(part 1 of 3)
# Autodesk Inventor assembly: Assembly1
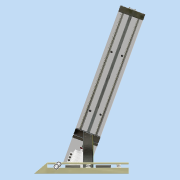
[picture p0: Inventor's stored thumbnail of the model, 180x180]
Saved by Autodesk Inventor 2021 (Build 250183000, 183)
## iProperties
Created: 2024-03-13
Part Number: Assembly1
Document SubType Name: Assembly
Designer: Nokia
Author: Nokia
## Documents named in this file (48)
- C:\Users\Nokia\Desktop\KP22\KP2\Assembly1.iam
- C:\Users\Nokia\Desktop\KP22\KP2\Plattform-Oberteil.ipt
- C:\Users\Nokia\Desktop\KP22\KP2\Spindel.ipt
- C:\Users\Nokia\Documents\Inventor\Content Center Files\R2021\en-US\DIN 711 SKF\DIN 711 SKF - SKF 51108.ipt
- C:\Users\Nokia\Documents\Inventor\Content Center Files\R2021\en-US\DIN 981\DIN 981 - KM 6.ipt
- C:\Users\Nokia\Documents\Inventor\Content Center Files\R2021\en-US\DIN 5406 Type MB_MBL (- DIN 981)\DIN 5406 - MB6.ipt
- C:\Users\Nokia\Documents\Inventor\Content Center Files\R2021\en-US\DIN 625 SKF(5)\DIN 625 SKF - SKF 6206-2RS1.ipt
- C:\Users\Nokia\Desktop\KP22\KP2\Festlagertopf.ipt
- C:\Users\Nokia\Desktop\KP22\KP2\Deckel.ipt
- C:\Users\Nokia\Desktop\KP22\KP2\Deckelscheibe.ipt
- C:\Users\Nokia\Desktop\KP22\KP2\Plattform-Unterteil.ipt
- C:\Users\Nokia\Desktop\KP22\KP2\Verbindungsplatte.ipt
- C:\Users\Nokia\Documents\Inventor\Content Center Files\R2021\en-US\DIN 625 SKF(5)\DIN 625 SKF - SKF 6005-2RSH.ipt
- C:\Users\Nokia\Documents\Inventor\Content Center Files\R2021\en-US\DIN 5406 Type MB_MBL (- DIN 981)\DIN 5406 - MB5.ipt
- C:\Users\Nokia\Documents\Inventor\Content Center Files\R2021\en-US\DIN 981\DIN 981 - KM 5.ipt
- C:\Users\Nokia\Desktop\KP22\KP2\Loslagertopf.ipt
- C:\Users\Nokia\Desktop\KP22\KP2\Verfahrschlitten.ipt
- C:\Users\Nokia\Desktop\KP22\KP2\Federwellen-Gleitlager.ipt
- C:\Users\Nokia\Desktop\KP22\KP2\Federführungswellen.ipt
- C:\Users\Nokia\Desktop\KP22\KP2\Hülle des Plattform-Oberteils.ipt
- C:\Users\Nokia\Desktop\KP22\KP2\Hülle des Plattform-Unterteils.ipt
- C:\Users\Nokia\Documents\Inventor\Content Center Files\R2021\en-US\DIN 931-1\DIN 931-1 - M6 x 30.ipt
- C:\Users\Nokia\Documents\Inventor\Content Center Files\R2021\en-US\DIN 125-1  B\DIN 125-1 - B 6,4.ipt
- C:\Users\Nokia\Documents\Inventor\Content Center Files\R2021\en-US\DIN 931-1\DIN 931-1 - M8 x 50.ipt
- C:\Users\Nokia\Documents\Inventor\Content Center Files\R2021\en-US\DIN 125-1  B\DIN 125-1 - B 8,4.ipt
- C:\Users\Nokia\Documents\Inventor\Content Center Files\R2021\en-US\DIN 931-1\DIN 931-1 - M6 x 50.ipt
- C:\Users\Nokia\Desktop\KP22\KP2\Gewindemutter.ipt
- C:\Users\Nokia\Documents\Inventor\Content Center Files\R2021\en-US\DIN 125-1  B\DIN 125-1 - B 5,3.ipt
- C:\Users\Nokia\Documents\Inventor\Content Center Files\R2021\en-US\DIN 931-1\DIN 931-1 - M5 x 25.ipt
- C:\Users\Nokia\Desktop\KP22\KP2\Führung.ipt
- C:\Users\Nokia\Documents\Inventor\Content Center Files\R2021\en-US\DIN 931-1\DIN 931-1 - M5 x 50.ipt
- C:\Users\Nokia\Desktop\KP22\KP2\Führungsgleitlager.ipt
- C:\Users\Nokia\Desktop\KP22\KP2\Schutzpuffer.ipt
- C:\Users\Nokia\Desktop\KP22\KP2\Grundplatte.ipt
- C:\Users\Nokia\Documents\Inventor\Content Center Files\R2021\en-US\DIN 125-1  B\DIN 125-1 - B 13.ipt
- C:\Users\Nokia\Documents\Inventor\Content Center Files\R2021\en-US\DIN 931-1\DIN 931-1 - M12 x 70.ipt
- C:\Users\Nokia\Desktop\KP22\KP2\Elektromotor.ipt
- C:\Users\Nokia\Desktop\KP22\KP2\Ausgleichskupplung.iam
- C:\Users\Nokia\Documents\Inventor\Content Center Files\R2021\en-US\DIN 912\DIN 912 - M12 x 1,75 x 50 x 45,625.ipt
- C:\Users\Nokia\Documents\Inventor\Content Center Files\R2021\en-US\DIN 6915\DIN 6915 - M12.ipt
- C:\Users\Nokia\Documents\Inventor\Content Center Files\R2021\en-US\DIN 6885-1 A\DIN 6885 - A 4 x 4 x 12.ipt
- C:\Users\Nokia\Documents\Inventor\Content Center Files\R2021\en-US\DIN EN ISO 4026\DIN EN ISO 4026 - M8 x 10.ipt
- C:\Users\Nokia\Desktop\KP22\KP2\Rubber Kupplung.ipt
- C:\Users\Nokia\Desktop\KP22\KP2\Elektrischer Schalter.ipt
- C:\Users\Nokia\Desktop\KP22\KP2\Wand.ipt
- C:\Users\Nokia\Desktop\KP22\KP2\Compress Spring11.ipt
- C:\Users\Nokia\Documents\Inventor\Content Center Files\R2021\en-US\DIN 931-1\DIN 931-1 - M12 x 55.ipt
- C:\Users\Nokia\Documents\Inventor\Content Center Files\R2021\en-US\DIN 931-1\DIN 931-1 - M8 x 45.ipt
## Components (277 placed, 47 different names)
1. Plattform-Oberteil:1 — Mate:60, Mate:61, Mate:62, Mate:63, Mate:64, Mate:65, Mate:66, Mate:67, Mate:68, Mate:69, Mate:70, Mate:71, Mate:85, Mate:86, Mate:87, Mate:88, Mate:89, Mate:90, Mate:91, Mate:92, Mate:93, Mate:94, Mate:95, Mate:96, Mate:97, Angle:13, Angle:14, Angle:15, Angle:16, Angle:17, Mate:122, Mate:123, Mate:124, Mate:125, Mate:126, Mate:127, Mate:146, Mate:147, Mate:153, Mate:154, Mate:191, Mate:192, Mate:193, Mate:194, Mate:195, Mate:196, Mate:197, Mate:198, Mate:199, Mate:200, Mate:201, Mate:202, Mate:203, Mate:204, Mate:205, Mate:206, Mate:207, Mate:223, Mate:224, Mate:225, Mate:226, Mate:227, Mate:497, Mate:645, Mate:646, Mate:647, Mate:648, Mate:649, Mate:650
2. DIN 711 SKF SKF 51108:1 — Mate:10, Mate:11, Mate:18, Mate:655
3. DIN 625 SKF- with two RS1 seals SKF 6206-2RS1:1 — Mate:3, Mate:4, Mate:20, Mate:651, Mate:654
4. Spindel:1 — Mate:3, Mate:4, Mate:10, Mate:11, Mate:13, Mate:14, Mate:17, Mate:19, Mate:21, Mate:46, Mate:47, Mate:48, Mate:50, Angle:5, Mate:52, Mate:55, Mate:548, Mate:551, Mate:552, Mate:553, Angle:21, Mate:654, Mate:655, Mate:656
5. DIN 981 KM 6:1 — Mate:16, Mate:17, Angle:2
6. DIN 5406 Type MB/MBL (->DIN 981) MB6:1 — Mate:13, Mate:14, Mate:16, Mate:651
7. Festlagertopf:1 — Mate:18, Mate:19, Angle:2, Angle:4, Mate:272, Mate:321, Mate:322, Mate:323, Mate:324, Mate:337, Mate:338, Mate:339, Mate:340, Mate:341, Mate:342, Mate:343, Mate:344, Mate:345, Mate:346, Mate:347, Mate:348, Flush:4, Mate:447, Mate:473, Mate:474, Mate:475, Mate:476, Mate:477, Mate:478, Mate:479, Angle:21
8. Deckel:1 — Mate:20, Mate:21, Mate:28, Mate:29, Mate:30, Mate:31, Mate:32, Mate:33, Mate:266, Mate:267, Mate:268, Mate:269, Mate:270, Mate:271
9. Deckelscheibe:1 — Mate:22, Mate:23, Mate:31
10. Deckelscheibe:2 — Mate:22, Mate:23, Mate:28
11. Deckelscheibe:3 — Mate:33
12. Deckelscheibe:4 — Mate:30
13. Deckelscheibe:5 — Mate:32
14. Deckelscheibe:6 — Mate:29
15. Plattform-Unterteil:1 — Mate:36, Mate:37, Mate:38, Mate:72, Mate:73, Mate:74, Mate:75, Mate:76, Mate:77, Mate:78, Mate:79, Mate:80, Mate:81, Mate:82, Mate:83, Mate:116, Mate:117, Mate:118, Mate:119, Mate:120, Mate:121, Mate:134, Mate:135, Mate:136, Mate:137, Mate:138, Mate:139, Mate:236, Mate:237, Mate:238, Mate:239, Mate:242, Mate:243, Mate:497, Mate:617, Mate:618, Flush:10, Flush:11, Flush:12, Flush:13, Angle:136, Angle:154, Angle:156, Angle:158, Angle:162, Angle:164, Angle:176
16. Verbindungsplatte:1 — Mate:36, Mate:37, Mate:38, Mate:53, Mate:56, Mate:57, Mate:58, Mate:59, Mate:240, Mate:241, Mate:252, Mate:253, Mate:254, Mate:255, Mate:256, Mate:257, Mate:258, Mate:259
17. DIN 625 SKF- with two RS1 seals SKF 6005-2RSH:1 — Mate:40, Mate:41, Mate:46, Mate:47, Mate:652, Mate:656
18. DIN 981 KM 5:1 — Mate:51, Angle:5, Mate:52
19. DIN 5406 Type MB/MBL (->DIN 981) MB5:1 — Mate:48, Mate:50, Mate:51, Mate:652
20. Loslagertopf:1 — Mate:40, Mate:41, Angle:4, Angle:6, Mate:492, Mate:493, Mate:494, Mate:495, Mate:657
21. Verfahrschlitten:1 — Mate:53, Angle:6, Mate:55, Mate:56, Mate:57, Mate:58, Mate:59, Mate:275, Mate:276, Mate:277, Mate:278, Mate:279, Mate:301, Mate:302, Mate:303, Mate:304, Mate:305, Mate:311, Mate:313, Mate:314, Mate:315, Mate:316, Mate:389, Mate:390, Mate:393, Mate:394, Mate:404, Mate:405, Mate:406, Mate:407, Mate:408, Mate:409, Mate:410, Mate:411, Mate:412, Mate:413, Mate:414, Mate:415, Mate:418, Mate:420, Mate:421, Mate:422, Mate:423, Mate:424, Mate:425, Mate:426, Mate:427, Mate:428, Mate:429, Mate:430, Mate:501, Mate:502, Angle:18, Angle:19, Flush:5, Flush:6, Flush:7, Flush:8, Mate:504, Angle:84, Angle:85, Angle:102, Angle:103, Angle:107, Angle:112, Angle:117, Angle:122, Angle:126, Angle:127
22. Federwellen-Gleitlager:1 — Mate:60, Mate:66
23. Federwellen-Gleitlager:2 — Mate:61, Mate:67
24. Federwellen-Gleitlager:3 — Mate:65, Mate:71
25. Federwellen-Gleitlager:4 — Mate:64, Mate:70
26. Federwellen-Gleitlager:5 — Mate:62, Mate:69
27. Federwellen-Gleitlager:6 — Mate:63, Mate:68
28. Federwellen-Gleitlager:7 — Mate:72, Mate:79, Mate:85
29. Federwellen-Gleitlager:8 — Mate:75, Mate:81
30. Federwellen-Gleitlager:9 — Mate:74, Mate:80
31. Federwellen-Gleitlager:10 — Mate:77, Mate:82, Mate:496
32. Federwellen-Gleitlager:11 — Mate:76, Mate:83
33. Federwellen-Gleitlager:12 — Mate:73, Mate:78
34. Federführungswellen:1 — Mate:87, Mate:95, Mate:115, Mate:129, Mate:143, Mate:208, Mate:209, Mate:210, Mate:644
35. Federführungswellen:2 — Mate:86, Mate:96, Mate:114, Mate:128, Mate:142, Mate:149, Mate:639
36. Federführungswellen:3 — Mate:88, Mate:97, Mate:112, Mate:131, Mate:144, Mate:211, Mate:212, Mate:213, Mate:643
37. Federführungswellen:4 — Mate:89, Mate:94, Mate:113, Mate:130, Mate:141, Mate:214, Mate:215, Mate:216, Mate:640
38. Federführungswellen:5 — Mate:90, Mate:92, Mate:98, Mate:99, Mate:132, Mate:140, Mate:217, Mate:218, Mate:219, Mate:496, Mate:641
39. Federführungswellen:6 — Mate:91, Mate:93, Mate:111, Mate:133, Mate:145, Mate:220, Mate:221, Mate:222, Mate:642
40. DIN 981 KM 6:3 — Mate:101, Mate:102, Angle:8, Mate:116, Angle:155
41. DIN 981 KM 6:4 — Mate:98, Mate:100, Angle:7, Mate:117, Angle:157
42. DIN 981 KM 6:6 — Mate:99, Mate:100, Angle:7, Angle:156, Angle:157
43. DIN 981 KM 6:7 — Mate:101, Mate:102, Angle:8, Mate:111, Angle:17, Angle:154, Angle:155
44. DIN 981 KM 6:8 — Mate:121, Angle:163
45. DIN 981 KM 6:9 — Mate:114, Angle:13, Angle:162, Angle:163
46. DIN 981 KM 6:10 — Mate:119, Angle:159
47. DIN 981 KM 6:11 — Mate:112, Angle:16, Angle:158, Angle:159, Angle:160
48. DIN 981 KM 6:12 — Mate:118, Angle:161
49. DIN 981 KM 6:13 — Mate:113, Angle:15, Angle:160, Angle:161
50. DIN 981 KM 6:14 — Mate:120, Angle:165
51. DIN 981 KM 6:15 — Mate:115, Angle:14, Angle:164, Angle:165
52. Hülle des Plattform-Oberteils:1 — Mate:125, Mate:130
53. Hülle des Plattform-Oberteils:2 — Mate:126, Mate:132
54. Hülle des Plattform-Oberteils:3 — Mate:127, Mate:133
55. Hülle des Plattform-Oberteils:4 — Mate:124, Mate:131
56. Hülle des Plattform-Oberteils:5 — Mate:122, Mate:128
57. Hülle des Plattform-Oberteils:6 — Mate:123, Mate:129
58. Hülle des Plattform-Unterteils:1 — Mate:134, Mate:142
59. Hülle des Plattform-Unterteils:2 — Mate:135, Mate:143
60. Hülle des Plattform-Unterteils:3 — Mate:136, Mate:141
61. Hülle des Plattform-Unterteils:4 — Mate:137, Mate:144
62. Hülle des Plattform-Unterteils:5 — Mate:138, Mate:140
63. Hülle des Plattform-Unterteils:6 — Mate:139, Mate:145
64. DIN 125-1 B B 6,4:1 — Mate:146, Mate:147, Mate:148, Mate:150
65. DIN 931-1 - replaced by DIN EN 24014 M6 x 30:1 — Mate:148, Mate:149, Mate:150, Angle:141
66. DIN 125-1 B B 6,4:2 — Mate:153
67. DIN 931-1 - replaced by DIN EN 24014 M6 x 30:2 — Mate:154, Angle:139, Angle:140, Angle:141, Angle:142
68. DIN 125-1 B B 6,4:4 — Mate:197
69. DIN 931-1 - replaced by DIN EN 24014 M6 x 30:4 — Mate:212, Mate:225, Angle:147
70. DIN 125-1 B B 6,4:5 — Mate:202
71. DIN 931-1 - replaced by DIN EN 24014 M6 x 30:5 — Mate:217, Mate:227, Angle:148, Angle:150, Angle:151
72. DIN 125-1 B B 6,4:7 — Mate:198
73. DIN 931-1 - replaced by DIN EN 24014 M6 x 30:7 — Mate:215, Angle:142, Angle:143
74. DIN 125-1 B B 6,4:8 — Mate:200, Mate:224
75. DIN 931-1 - replaced by DIN EN 24014 M6 x 30:8 — Mate:214, Angle:143, Angle:144
76. DIN 125-1 B B 6,4:9 — Mate:204
77. DIN 931-1 - replaced by DIN EN 24014 M6 x 30:9 — Mate:220, Angle:153
78. DIN 125-1 B B 6,4:10 — Mate:195
79. DIN 931-1 - replaced by DIN EN 24014 M6 x 30:10 — Mate:213, Angle:145, Angle:146, Angle:148
80. DIN 125-1 B B 6,4:11 — Mate:196
81. DIN 931-1 - replaced by DIN EN 24014 M6 x 30:11 — Mate:211, Angle:146, Angle:147
82. DIN 125-1 B B 6,4:12 — Mate:206
83. DIN 931-1 - replaced by DIN EN 24014 M6 x 30:12 — Mate:222, Angle:151, Angle:152, Angle:153
84. DIN 125-1 B B 6,4:13 — Mate:201
85. DIN 931-1 - replaced by DIN EN 24014 M6 x 30:13 — Mate:218, Angle:184
86. DIN 125-1 B B 6,4:14 — Mate:205
87. DIN 931-1 - replaced by DIN EN 24014 M6 x 30:14 — Mate:221, Mate:226, Angle:152
88. DIN 125-1 B B 6,4:15 — Mate:203
89. DIN 931-1 - replaced by DIN EN 24014 M6 x 30:15 — Mate:219, Angle:150, Angle:184
90. DIN 125-1 B B 6,4:16 — Mate:192
91. DIN 931-1 - replaced by DIN EN 24014 M6 x 30:16 — Mate:210, Angle:138, Angle:139
92. DIN 125-1 B B 6,4:17 — Mate:194, Mate:207
93. DIN 931-1 - replaced by DIN EN 24014 M6 x 30:17 — Angle:140
94. DIN 125-1 B B 6,4:18 — Mate:199
95. DIN 931-1 - replaced by DIN EN 24014 M6 x 30:18 — Mate:216, Angle:144, Angle:145
96. DIN 125-1 B B 6,4:19 — Mate:191
97. DIN 931-1 - replaced by DIN EN 24014 M6 x 30:19 — Mate:208, Mate:223, Angle:136, Angle:137
98. DIN 125-1 B B 6,4:20 — Mate:193
99. DIN 931-1 - replaced by DIN EN 24014 M6 x 30:20 — Mate:209, Angle:137, Angle:138
100. DIN 931-1 - replaced by DIN EN 24014 M8 x 45:1 — Mate:228, Mate:229, Mate:243, Angle:175, Angle:180, Angle:181, Angle:182, Angle:183
101. DIN 125-1 B B 8,4:1 — Mate:228, Mate:229, Mate:236
102. DIN 931-1 - replaced by DIN EN 24014 M8 x 45:2 — Mate:242, Angle:175, Angle:181
103. DIN 125-1 B B 8,4:2 — Mate:238
104. DIN 931-1 - replaced by DIN EN 24014 M8 x 45:3 — Mate:240, Angle:183
105. DIN 125-1 B B 8,4:3 — Mate:239
106. DIN 931-1 - replaced by DIN EN 24014 M8 x 45:4 — Mate:241, Angle:182
107. DIN 125-1 B B 8,4:4 — Mate:237
108. DIN 931-1 - replaced by DIN EN 24014 M8 x 50:5 — Mate:259, Angle:178
109. DIN 125-1 B B 8,4:5 — Mate:255
110. DIN 931-1 - replaced by DIN EN 24014 M8 x 50:6 — Mate:258, Angle:179, Angle:180
111. DIN 125-1 B B 8,4:6 — Mate:254
112. DIN 931-1 - replaced by DIN EN 24014 M8 x 50:7 — Mate:257, Angle:177, Angle:178, Angle:179
113. DIN 125-1 B B 8,4:7 — Mate:253
114. DIN 931-1 - replaced by DIN EN 24014 M8 x 50:8 — Mate:256, Angle:176, Angle:177
115. DIN 125-1 B B 8,4:8 — Mate:252
116. DIN 931-1 - replaced by DIN EN 24014 M6 x 50:3 — Mate:270, Angle:32
117. DIN 125-1 B B 6,4:23 — Mate:268
118. DIN 931-1 - replaced by DIN EN 24014 M6 x 50:2 — Mate:269, Mate:272, Angle:33
119. DIN 125-1 B B 6,4:21 — Mate:266
120. DIN 931-1 - replaced by DIN EN 24014 M6 x 50:1 — Mate:271, Angle:28, Angle:31
121. DIN 125-1 B B 6,4:22 — Mate:267
122. DIN 931-1 - replaced by DIN EN 24014 M5 x 25:1 — Mate:279, Mate:312, Angle:111
123. DIN 125-1 B B 5,3:2 — Mate:280
124. Gewindemutter:1 — Mate:275, Mate:276, Mate:280, Mate:312, Mate:317, Mate:318, Mate:319, Mate:320
125. Gewindemutter:2 — Mate:277, Mate:278, Mate:306, Mate:307, Mate:308, Mate:309, Mate:310
126. DIN 931-1 - replaced by DIN EN 24014 M5 x 25:2 — Mate:320, Angle:109, Angle:111
127. DIN 125-1 B B 5,3:3 — Mate:316
128. DIN 931-1 - replaced by DIN EN 24014 M5 x 25:3 — Mate:318, Angle:108
129. DIN 125-1 B B 5,3:4 — Mate:315
130. DIN 931-1 - replaced by DIN EN 24014 M5 x 25:4 — Mate:308, Angle:126
131. DIN 125-1 B B 5,3:5 — Mate:305
132. DIN 931-1 - replaced by DIN EN 24014 M5 x 25:5 — Mate:319, Angle:107, Angle:108, Angle:109, Angle:110
133. DIN 125-1 B B 5,3:6 — Mate:313
134. DIN 931-1 - replaced by DIN EN 24014 M5 x 25:6 — Mate:307, Angle:125
135. DIN 125-1 B B 5,3:7 — Mate:304
136. DIN 931-1 - replaced by DIN EN 24014 M5 x 25:7 — Mate:317, Angle:110
137. DIN 125-1 B B 5,3:8 — Mate:314
138. DIN 931-1 - replaced by DIN EN 24014 M5 x 25:8 — Mate:309, Mate:311, Angle:124
139. DIN 125-1 B B 5,3:9 — Mate:301
140. DIN 931-1 - replaced by DIN EN 24014 M5 x 25:9 — Mate:310, Angle:123
141. DIN 125-1 B B 5,3:10 — Mate:302
142. DIN 931-1 - replaced by DIN EN 24014 M5 x 25:11 — Mate:306, Angle:122, Angle:123, Angle:124, Angle:125
143. DIN 125-1 B B 5,3:12 — Mate:303
144. Führung:1 — Mate:321, Mate:323, Mate:417, Mate:505, Mate:653
145. Führung:2 — Mate:322, Mate:324, Mate:391, Mate:416
146. DIN 931-1 - replaced by DIN EN 24014 M5 x 50:4 — Mate:345, Angle:25
147. DIN 125-1 B B 5,3:14 — Mate:337
148. DIN 931-1 - replaced by DIN EN 24014 M5 x 50:1 — Mate:347, Angle:30, Mate:653
149. DIN 125-1 B B 5,3:16 — Mate:338
150. DIN 931-1 - replaced by DIN EN 24014 M5 x 50:2 — Mate:348, Angle:29
151. DIN 125-1 B B 5,3:17 — Mate:340
152. DIN 931-1 - replaced by DIN EN 24014 M5 x 50:5 — Mate:343, Angle:26
153. DIN 125-1 B B 5,3:18 — Mate:342
154. DIN 931-1 - replaced by DIN EN 24014 M5 x 50:6 — Mate:344, Angle:27
155. DIN 125-1 B B 5,3:19 — Mate:339
156. DIN 931-1 - replaced by DIN EN 24014 M5 x 50:3 — Mate:346
157. DIN 125-1 B B 5,3:20 — Mate:341
158. DIN 931-1 - replaced by DIN EN 24014 M5 x 25:12 — Mate:438, Angle:104, Angle:105
159. DIN 125-1 B B 5,3:21 — Mate:421
160. Führungsgleitlager:1 — Mate:417, Mate:418, Mate:431, Mate:432, Mate:433, Mate:434, Mate:440
161. Führungsgleitlager:2 — Mate:415, Mate:416, Mate:420, Mate:435, Mate:436, Mate:437, Mate:438, Mate:439
162. Führungsgleitlager:3 — Mate:389, Mate:393, Mate:395, Mate:396, Mate:397, Mate:398, Mate:399, Mate:400, Mate:401, Mate:402, Mate:403, Mate:505
163. Führungsgleitlager:4 — Mate:390, Mate:391, Mate:394
164. DIN 931-1 - replaced by DIN EN 24014 M5 x 25:13 — Mate:437, Angle:103, Angle:106
165. DIN 125-1 B B 5,3:22 — Mate:428
166. DIN 931-1 - replaced by DIN EN 24014 M5 x 25:14 — Mate:410, Angle:128
167. DIN 125-1 B B 5,3:23 — Mate:401
168. DIN 931-1 - replaced by DIN EN 24014 M5 x 25:15 — Mate:413, Angle:118
169. DIN 125-1 B B 5,3:24 — Mate:396
170. DIN 931-1 - replaced by DIN EN 24014 M5 x 25:16 — Mate:409, Angle:130
171. DIN 125-1 B B 5,3:25 — Mate:404
172. DIN 931-1 - replaced by DIN EN 24014 M5 x 25:17 — Mate:435, Angle:105
173. DIN 125-1 B B 5,3:26 — Mate:424
174. DIN 931-1 - replaced by DIN EN 24014 M5 x 25:18 — Mate:408, Angle:121
175. DIN 125-1 B B 5,3:27 — Mate:400
176. DIN 931-1 - replaced by DIN EN 24014 M5 x 25:19 — Mate:405, Angle:119
177. DIN 125-1 B B 5,3:28 — Mate:398
178. DIN 931-1 - replaced by DIN EN 24014 M5 x 25:20 — Mate:407, Angle:117, Angle:118, Angle:119, Angle:120, Angle:121
179. DIN 125-1 B B 5,3:29 — Mate:399
180. DIN 931-1 - replaced by DIN EN 24014 M5 x 25:21 — Mate:412, Angle:129
181. DIN 125-1 B B 5,3:30 — Mate:403
182. DIN 931-1 - replaced by DIN EN 24014 M5 x 25:22 — Mate:406, Angle:120
183. DIN 125-1 B B 5,3:31 — Mate:402
184. DIN 931-1 - replaced by DIN EN 24014 M5 x 25:23 — Mate:411, Angle:131
185. DIN 125-1 B B 5,3:32 — Mate:397
186. DIN 931-1 - replaced by DIN EN 24014 M5 x 25:24 — Mate:439, Angle:102, Angle:104
187. DIN 125-1 B B 5,3:33 — Mate:427
188. DIN 931-1 - replaced by DIN EN 24014 M5 x 25:25 — Mate:436, Angle:106
189. DIN 125-1 B B 5,3:34 — Mate:422
190. DIN 931-1 - replaced by DIN EN 24014 M5 x 25:26 — Mate:432, Mate:504, Angle:115
191. DIN 125-1 B B 5,3:35 — Mate:430
192. DIN 931-1 - replaced by DIN EN 24014 M5 x 25:27 — Mate:433, Angle:116
193. DIN 125-1 B B 5,3:36 — Mate:423
194. DIN 931-1 - replaced by DIN EN 24014 M5 x 25:28 — Mate:414, Angle:127, Angle:128, Angle:129, Angle:130, Angle:131
195. DIN 125-1 B B 5,3:37 — Mate:395
196. DIN 931-1 - replaced by DIN EN 24014 M5 x 25:29 — Mate:434, Angle:113
197. DIN 125-1 B B 5,3:38 — Mate:425
198. DIN 931-1 - replaced by DIN EN 24014 M5 x 25:30 — Mate:440, Angle:112, Angle:113, Angle:114, Angle:115, Angle:116
199. DIN 125-1 B B 5,3:39 — Mate:429
200. DIN 931-1 - replaced by DIN EN 24014 M5 x 25:31 — Mate:431, Angle:114
201. DIN 125-1 B B 5,3:40 — Mate:426
202. Grundplatte:1 — Flush:4, Mate:447, Mate:465, Mate:466, Mate:467, Mate:468, Mate:469, Mate:470, Mate:471, Mate:472, Mate:488, Mate:489, Mate:490, Mate:491, Mate:499, Mate:500, Angle:20, Flush:9, Mate:520, Mate:521, Mate:522, Mate:523, Mate:524, Mate:525, Mate:531, Mate:532, Mate:546, Mate:547, Mate:619, Mate:628, Mate:629, Mate:630, Mate:631, Mate:632, Mate:633, Mate:634, Mate:635, Angle:25, Angle:26, Angle:27, Angle:28, Angle:29, Angle:30, Angle:31, Angle:32, Angle:33, Angle:34, Angle:35, Angle:36, Angle:37, Angle:38, Angle:39, Angle:40, Angle:41, Angle:42, Angle:43, Angle:44, Angle:45, Angle:86, Angle:87, Angle:88, Angle:89, Angle:90, Angle:91, Angle:92, Angle:93, Angle:94, Angle:95, Angle:96, Angle:97, Angle:166, Angle:167
203. DIN 931-1 - replaced by DIN EN 24014 M12 x 70:1 — Mate:478, Angle:92
204. DIN 125-1 B B 13:1 — Mate:465
205. DIN 931-1 - replaced by DIN EN 24014 M12 x 70:2 — Mate:500, Angle:91
206. DIN 125-1 B B 13:2 — Mate:466
207. DIN 931-1 - replaced by DIN EN 24014 M12 x 70:3 — Mate:473, Angle:97
208. DIN 125-1 B B 13:3 — Mate:467
209. DIN 931-1 - replaced by DIN EN 24014 M12 x 70:4 — Mate:474, Angle:96
210. DIN 125-1 B B 13:4 — Mate:468
211. DIN 931-1 - replaced by DIN EN 24014 M12 x 70:5 — Mate:475, Angle:95
212. DIN 125-1 B B 13:5 — Mate:469
213. DIN 931-1 - replaced by DIN EN 24014 M12 x 70:6 — Mate:476, Angle:94
214. DIN 125-1 B B 13:6 — Mate:470
215. DIN 931-1 - replaced by DIN EN 24014 M12 x 70:7 — Mate:477, Angle:93
216. DIN 125-1 B B 13:7 — Mate:471
217. DIN 931-1 - replaced by DIN EN 24014 M12 x 70:8 — Mate:479, Angle:90
218. DIN 125-1 B B 13:8 — Mate:472
219. DIN 931-1 - replaced by DIN EN 24014 M12 x 70:9 — Mate:494, Angle:88
220. DIN 125-1 B B 13:9 — Mate:489
221. DIN 931-1 - replaced by DIN EN 24014 M12 x 70:10 — Mate:492, Angle:86
222. DIN 125-1 B B 13:10 — Mate:488
223. DIN 931-1 - replaced by DIN EN 24014 M12 x 70:11 — Mate:493, Mate:499, Angle:82, Angle:83, Angle:87
224. DIN 125-1 B B 13:11 — Mate:490
225. DIN 931-1 - replaced by DIN EN 24014 M12 x 70:12 — Mate:495, Angle:89
226. DIN 125-1 B B 13:12 — Mate:491
227. Schutzpuffer:1 — Mate:502, Angle:18, Flush:5, Flush:6, Mate:657
228. Schutzpuffer:2 — Mate:501, Angle:19, Flush:7, Flush:8
229. Elektromotor:1 — Angle:20, Flush:9, Mate:526, Mate:527, Mate:528, Mate:529, Mate:530, Mate:533, Mate:534, Mate:535, Mate:536, Mate:537, Mate:538, Mate:539, Mate:547, Mate:548, Mate:549, Mate:550, Mate:636, Mate:637, Mate:638
230. Ausgleichskupplung:1 [sub-assembly] — Mate:549, Mate:550, Angle:22, Mate:561, Mate:562
231. DIN 912 - replaced by DIN EN ISO 4762 M12 x 50:1 — Mate:508, Mate:509, Mate:530, Mate:544, Angle:37
232. DIN 125-1 B B 13:13 — Mate:508, Mate:509, Mate:525
233. DIN 912 - replaced by DIN EN ISO 4762 M12 x 50:2 — Mate:529, Mate:543, Angle:39
234. DIN 125-1 B B 13:14 — Mate:524
235. DIN 912 - replaced by DIN EN ISO 4762 M12 x 50:3 — Mate:527, Mate:540, Angle:45
236. DIN 125-1 B B 13:15 — Mate:520, Mate:522
237. DIN 912 - replaced by DIN EN ISO 4762 M12 x 50:4 — Mate:533, Mate:545, Angle:38
238. DIN 125-1 B B 13:16 — Mate:532
239. DIN 912 - replaced by DIN EN ISO 4762 M12 x 50:5 — Mate:528, Mate:541, Angle:44
240. DIN 125-1 B B 13:17 — Mate:521, Mate:523
241. DIN 912 - replaced by DIN EN ISO 4762 M12 x 50:6 — Mate:526, Mate:542, Mate:546, Angle:43
242. DIN 125-1 B B 13:18 — Mate:531
243. DIN 125-1 B B 13:19 — Mate:539, Mate:541, Insert:5
244. DIN 125-1 B B 13:20 — Mate:538, Mate:542, Insert:4
245. DIN 125-1 B B 13:21 — Mate:537, Mate:543, Insert:1
246. DIN 125-1 B B 13:22 — Mate:536, Mate:540, Insert:6
247. DIN 125-1 B B 13:23 — Mate:535, Mate:545, Insert:3
248. DIN 125-1 B B 13:24 — Mate:534, Mate:544, Insert:2
249. DIN 6915 M12:1 — Insert:1, Angle:36
250. DIN 6915 M12:2 — Insert:2, Angle:35
251. DIN 6915 M12:3 — Insert:3, Angle:34
252. DIN 6915 M12:4 — Insert:4, Angle:42
253. DIN 6915 M12:5 — Insert:5, Angle:41
254. DIN 6915 M12:6 — Insert:6, Angle:40
255. DIN 6885-1 A A 4 x 4 x 12:2 — Mate:563, Mate:636, Mate:637, Mate:638, Angle:23
256. DIN 6885-1 A A 4 x 4 x 12:1 — Mate:551, Mate:552, Mate:553, Angle:22, Mate:564, Angle:24
257. DIN EN ISO 4026 M8 x 10:1 — Mate:557, Mate:559, Mate:562, Angle:83
258. DIN EN ISO 4026 M8 x 10:2 — Mate:558, Mate:560, Mate:561, Angle:82
259. Rubber Kupplung:1 — Mate:557, Mate:559, Mate:563, Angle:23
260. Rubber Kupplung:2 — Mate:558, Mate:560, Mate:564, Angle:24
261. Elektrischer Schalter:1 — Mate:617, Flush:11, Flush:13
262. Elektrischer Schalter:2 — Mate:618, Flush:10, Flush:12
263. Wand:1 — Mate:619
264. DIN 931-1 - replaced by DIN EN 24014 M12 x 55:4 — Mate:632, Angle:166
265. DIN 125-1 B B 13:26 — Mate:631
266. DIN 931-1 - replaced by DIN EN 24014 M12 x 55:3 — Mate:633, Angle:167
267. DIN 125-1 B B 13:25 — Mate:630
268. DIN 931-1 - replaced by DIN EN 24014 M12 x 55:1 — Mate:635, Angle:85
269. DIN 125-1 B B 13:28 — Mate:628
270. DIN 931-1 - replaced by DIN EN 24014 M12 x 55:2 — Mate:634, Angle:84
271. DIN 125-1 B B 13:27 — Mate:629
272. Compress Spring1:1 — Mate:639, Mate:645
273. Compress Spring1:2 — Mate:640, Mate:647
274. Compress Spring1:3 — Mate:641, Mate:648
275. Compress Spring1:4 — Mate:642, Mate:649
276. Compress Spring1:5 — Mate:643, Mate:650
277. Compress Spring1:6 — Mate:644, Mate:646
## Relationships (710: Mate 564, Angle 130, Flush 10, Insert 6)
- Mate:3: DIN 625 SKF- with two RS1 seals SKF 6206-2RS1:1 ↔ Spindel:1
- Mate:4: DIN 625 SKF- with two RS1 seals SKF 6206-2RS1:1 ↔ Spindel:1
- Mate:10: DIN 711 SKF SKF 51108:1 ↔ Spindel:1
- Mate:11: DIN 711 SKF SKF 51108:1 ↔ Spindel:1
- Mate:13: Spindel:1 ↔ DIN 5406 Type MB/MBL (->DIN 981) MB6:1
- Mate:14: Spindel:1 ↔ DIN 5406 Type MB/MBL (->DIN 981) MB6:1
- Mate:16: DIN 981 KM 6:1 ↔ DIN 5406 Type MB/MBL (->DIN 981) MB6:1
- Mate:17: Spindel:1 ↔ DIN 981 KM 6:1
- Mate:18: DIN 711 SKF SKF 51108:1 ↔ Festlagertopf:1
- Mate:19: Spindel:1 ↔ Festlagertopf:1
- Angle:2 (0 deg): DIN 981 KM 6:1 ↔ Festlagertopf:1
- Mate:20: DIN 625 SKF- with two RS1 seals SKF 6206-2RS1:1 ↔ Deckel:1
- Mate:21: Spindel:1 ↔ Deckel:1
- Mate:22: Deckelscheibe:1 ↔ Deckelscheibe:2
- Mate:23: Deckelscheibe:1 ↔ Deckelscheibe:2
- [Mate]: Deckelscheibe:3 ↔ Deckelscheibe:4
- [Mate]: Deckelscheibe:3 ↔ Deckelscheibe:4
- [Mate]: Deckelscheibe:5 ↔ Deckelscheibe:6
- [Mate]: Deckelscheibe:5 ↔ Deckelscheibe:6
- Mate:28: Deckel:1 ↔ Deckelscheibe:2
- Mate:29: Deckel:1 ↔ Deckelscheibe:6
- Mate:30: Deckel:1 ↔ Deckelscheibe:4
- Mate:31: Deckel:1 ↔ Deckelscheibe:1
- Mate:32: Deckel:1 ↔ Deckelscheibe:5
- Mate:33: Deckel:1 ↔ Deckelscheibe:3
- Mate:36: Plattform-Unterteil:1 ↔ Verbindungsplatte:1
- Mate:37: Plattform-Unterteil:1 ↔ Verbindungsplatte:1
- Mate:38: Plattform-Unterteil:1 ↔ Verbindungsplatte:1
- Mate:40: DIN 625 SKF- with two RS1 seals SKF 6005-2RSH:1 ↔ Loslagertopf:1
- Mate:41: DIN 625 SKF- with two RS1 seals SKF 6005-2RSH:1 ↔ Loslagertopf:1
- Angle:4 (0 deg): Festlagertopf:1 ↔ Loslagertopf:1
- Mate:46: Spindel:1 ↔ DIN 625 SKF- with two RS1 seals SKF 6005-2RSH:1
- Mate:47: Spindel:1 ↔ DIN 625 SKF- with two RS1 seals SKF 6005-2RSH:1
- Mate:48: Spindel:1 ↔ DIN 5406 Type MB/MBL (->DIN 981) MB5:1
- Mate:50: Spindel:1 ↔ DIN 5406 Type MB/MBL (->DIN 981) MB5:1
- Mate:51: DIN 981 KM 5:1 ↔ DIN 5406 Type MB/MBL (->DIN 981) MB5:1
- Angle:5 (0 deg): Spindel:1 ↔ DIN 981 KM 5:1
- Mate:52: Spindel:1 ↔ DIN 981 KM 5:1
- Mate:53: Verbindungsplatte:1 ↔ Verfahrschlitten:1
- Angle:6 (0 deg): Loslagertopf:1 ↔ Verfahrschlitten:1
- Mate:55: Spindel:1 ↔ Verfahrschlitten:1
- Mate:56: Verbindungsplatte:1 ↔ Verfahrschlitten:1
- Mate:57: Verbindungsplatte:1 ↔ Verfahrschlitten:1
- Mate:58: Verbindungsplatte:1 ↔ Verfahrschlitten:1
- Mate:59: Verbindungsplatte:1 ↔ Verfahrschlitten:1
- Mate:60: Plattform-Oberteil:1 ↔ Federwellen-Gleitlager:1
- Mate:61: Plattform-Oberteil:1 ↔ Federwellen-Gleitlager:2
- Mate:62: Plattform-Oberteil:1 ↔ Federwellen-Gleitlager:5
- Mate:63: Plattform-Oberteil:1 ↔ Federwellen-Gleitlager:6
- Mate:64: Plattform-Oberteil:1 ↔ Federwellen-Gleitlager:4
- Mate:65: Plattform-Oberteil:1 ↔ Federwellen-Gleitlager:3
- Mate:66: Plattform-Oberteil:1 ↔ Federwellen-Gleitlager:1
- Mate:67: Plattform-Oberteil:1 ↔ Federwellen-Gleitlager:2
- Mate:68: Plattform-Oberteil:1 ↔ Federwellen-Gleitlager:6
- Mate:69: Plattform-Oberteil:1 ↔ Federwellen-Gleitlager:5
- Mate:70: Plattform-Oberteil:1 ↔ Federwellen-Gleitlager:4
- Mate:71: Plattform-Oberteil:1 ↔ Federwellen-Gleitlager:3
- Mate:72: Plattform-Unterteil:1 ↔ Federwellen-Gleitlager:7
- Mate:73: Plattform-Unterteil:1 ↔ Federwellen-Gleitlager:12
- Mate:74: Plattform-Unterteil:1 ↔ Federwellen-Gleitlager:9
- Mate:75: Plattform-Unterteil:1 ↔ Federwellen-Gleitlager:8
- Mate:76: Plattform-Unterteil:1 ↔ Federwellen-Gleitlager:11
- Mate:77: Plattform-Unterteil:1 ↔ Federwellen-Gleitlager:10
- Mate:78: Plattform-Unterteil:1 ↔ Federwellen-Gleitlager:12
- Mate:79: Plattform-Unterteil:1 ↔ Federwellen-Gleitlager:7
- Mate:80: Plattform-Unterteil:1 ↔ Federwellen-Gleitlager:9
- Mate:81: Plattform-Unterteil:1 ↔ Federwellen-Gleitlager:8
- Mate:82: Plattform-Unterteil:1 ↔ Federwellen-Gleitlager:10
- Mate:83: Plattform-Unterteil:1 ↔ Federwellen-Gleitlager:11
- Mate:85: Plattform-Oberteil:1 ↔ Federwellen-Gleitlager:7
- Mate:86: Plattform-Oberteil:1 ↔ Federführungswellen:2
- Mate:87: Plattform-Oberteil:1 ↔ Federführungswellen:1
- Mate:88: Plattform-Oberteil:1 ↔ Federführungswellen:3
- Mate:89: Plattform-Oberteil:1 ↔ Federführungswellen:4
- Mate:90: Plattform-Oberteil:1 ↔ Federführungswellen:5
- Mate:91: Plattform-Oberteil:1 ↔ Federführungswellen:6
- Mate:92: Plattform-Oberteil:1 ↔ Federführungswellen:5
- Mate:93: Plattform-Oberteil:1 ↔ Federführungswellen:6
- Mate:94: Plattform-Oberteil:1 ↔ Federführungswellen:4
- Mate:95: Plattform-Oberteil:1 ↔ Federführungswellen:1
- Mate:96: Plattform-Oberteil:1 ↔ Federführungswellen:2
- Mate:97: Plattform-Oberteil:1 ↔ Federführungswellen:3
- Mate:98: Federführungswellen:5 ↔ DIN 981 KM 6:4
- Mate:99: Federführungswellen:5 ↔ DIN 981 KM 6:6
- Mate:100: DIN 981 KM 6:4 ↔ DIN 981 KM 6:6
- Angle:7 (0 deg): DIN 981 KM 6:4 ↔ DIN 981 KM 6:6
- Mate:101: DIN 981 KM 6:3 ↔ DIN 981 KM 6:7
- Mate:102: DIN 981 KM 6:3 ↔ DIN 981 KM 6:7
- Angle:8 (0 deg): DIN 981 KM 6:3 ↔ DIN 981 KM 6:7
- [Mate]: DIN 981 KM 6:8 ↔ DIN 981 KM 6:9
- [Mate]: DIN 981 KM 6:8 ↔ DIN 981 KM 6:9
- [Angle] (0 deg): DIN 981 KM 6:8 ↔ DIN 981 KM 6:9
- [Mate]: DIN 981 KM 6:10 ↔ DIN 981 KM 6:11
- [Mate]: DIN 981 KM 6:10 ↔ DIN 981 KM 6:11
- [Angle] (0 deg): DIN 981 KM 6:10 ↔ DIN 981 KM 6:11
- [Mate]: DIN 981 KM 6:12 ↔ DIN 981 KM 6:13
- [Mate]: DIN 981 KM 6:12 ↔ DIN 981 KM 6:13
- [Angle] (0 deg): DIN 981 KM 6:12 ↔ DIN 981 KM 6:13
- [Mate]: DIN 981 KM 6:14 ↔ DIN 981 KM 6:15
- [Mate]: DIN 981 KM 6:14 ↔ DIN 981 KM 6:15
- [Angle] (0 deg): DIN 981 KM 6:14 ↔ DIN 981 KM 6:15
- Mate:111: Federführungswellen:6 ↔ DIN 981 KM 6:7
- Mate:112: Federführungswellen:3 ↔ DIN 981 KM 6:11
- Mate:113: Federführungswellen:4 ↔ DIN 981 KM 6:13
- Mate:114: Federführungswellen:2 ↔ DIN 981 KM 6:9
- Mate:115: Federführungswellen:1 ↔ DIN 981 KM 6:15
- Angle:13 (0 deg): Plattform-Oberteil:1 ↔ DIN 981 KM 6:9
- Angle:14 (0 deg): Plattform-Oberteil:1 ↔ DIN 981 KM 6:15
- Angle:15 (0 deg): Plattform-Oberteil:1 ↔ DIN 981 KM 6:13
- Angle:16 (0 deg): Plattform-Oberteil:1 ↔ DIN 981 KM 6:11
- Angle:17 (0 deg): Plattform-Oberteil:1 ↔ DIN 981 KM 6:7
- Mate:116: Plattform-Unterteil:1 ↔ DIN 981 KM 6:3
- Mate:117: Plattform-Unterteil:1 ↔ DIN 981 KM 6:4
- Mate:118: Plattform-Unterteil:1 ↔ DIN 981 KM 6:12
- Mate:119: Plattform-Unterteil:1 ↔ DIN 981 KM 6:10
- Mate:120: Plattform-Unterteil:1 ↔ DIN 981 KM 6:14
- Mate:121: Plattform-Unterteil:1 ↔ DIN 981 KM 6:8
- Mate:122: Plattform-Oberteil:1 ↔ Hülle des Plattform-Oberteils:5
- Mate:123: Plattform-Oberteil:1 ↔ Hülle des Plattform-Oberteils:6
- Mate:124: Plattform-Oberteil:1 ↔ Hülle des Plattform-Oberteils:4
- Mate:125: Plattform-Oberteil:1 ↔ Hülle des Plattform-Oberteils:1
- Mate:126: Plattform-Oberteil:1 ↔ Hülle des Plattform-Oberteils:2
- Mate:127: Plattform-Oberteil:1 ↔ Hülle des Plattform-Oberteils:3
- Mate:128: Federführungswellen:2 ↔ Hülle des Plattform-Oberteils:5
- Mate:129: Federführungswellen:1 ↔ Hülle des Plattform-Oberteils:6
- Mate:130: Federführungswellen:4 ↔ Hülle des Plattform-Oberteils:1
- Mate:131: Federführungswellen:3 ↔ Hülle des Plattform-Oberteils:4
- Mate:132: Federführungswellen:5 ↔ Hülle des Plattform-Oberteils:2
- Mate:133: Federführungswellen:6 ↔ Hülle des Plattform-Oberteils:3
- Mate:134: Plattform-Unterteil:1 ↔ Hülle des Plattform-Unterteils:1
- Mate:135: Plattform-Unterteil:1 ↔ Hülle des Plattform-Unterteils:2
- Mate:136: Plattform-Unterteil:1 ↔ Hülle des Plattform-Unterteils:3
- Mate:137: Plattform-Unterteil:1 ↔ Hülle des Plattform-Unterteils:4
- Mate:138: Plattform-Unterteil:1 ↔ Hülle des Plattform-Unterteils:5
- Mate:139: Plattform-Unterteil:1 ↔ Hülle des Plattform-Unterteils:6
- Mate:140: Federführungswellen:5 ↔ Hülle des Plattform-Unterteils:5
- Mate:141: Federführungswellen:4 ↔ Hülle des Plattform-Unterteils:3
- Mate:142: Federführungswellen:2 ↔ Hülle des Plattform-Unterteils:1
- Mate:143: Federführungswellen:1 ↔ Hülle des Plattform-Unterteils:2
- Mate:144: Federführungswellen:3 ↔ Hülle des Plattform-Unterteils:4
- Mate:145: Federführungswellen:6 ↔ Hülle des Plattform-Unterteils:6
- Mate:146: Plattform-Oberteil:1 ↔ DIN 125-1 B B 6,4:1
- Mate:147: Plattform-Oberteil:1 ↔ DIN 125-1 B B 6,4:1
- Mate:148: DIN 125-1 B B 6,4:1 ↔ DIN 931-1 - replaced by DIN EN 24014 M6 x 30:1
- Mate:149: Federführungswellen:2 ↔ DIN 931-1 - replaced by DIN EN 24014 M6 x 30:1
- Mate:150: DIN 125-1 B B 6,4:1 ↔ DIN 931-1 - replaced by DIN EN 24014 M6 x 30:1
- [Mate]: DIN 125-1 B B 6,4:2 ↔ DIN 931-1 - replaced by DIN EN 24014 M6 x 30:2
- [Mate]: DIN 125-1 B B 6,4:2 ↔ DIN 931-1 - replaced by DIN EN 24014 M6 x 30:2
- Mate:153: Plattform-Oberteil:1 ↔ DIN 125-1 B B 6,4:2
- Mate:154: Plattform-Oberteil:1 ↔ DIN 931-1 - replaced by DIN EN 24014 M6 x 30:2
- [Mate]: DIN 125-1 B B 6,4:4 ↔ DIN 931-1 - replaced by DIN EN 24014 M6 x 30:4
- [Mate]: DIN 125-1 B B 6,4:4 ↔ DIN 931-1 - replaced by DIN EN 24014 M6 x 30:4
- [Mate]: DIN 125-1 B B 6,4:5 ↔ DIN 931-1 - replaced by DIN EN 24014 M6 x 30:5
- [Mate]: DIN 125-1 B B 6,4:5 ↔ DIN 931-1 - replaced by DIN EN 24014 M6 x 30:5
- [Mate]: DIN 125-1 B B 6,4:7 ↔ DIN 931-1 - replaced by DIN EN 24014 M6 x 30:7
- [Mate]: DIN 125-1 B B 6,4:7 ↔ DIN 931-1 - replaced by DIN EN 24014 M6 x 30:7
- [Mate]: DIN 125-1 B B 6,4:8 ↔ DIN 931-1 - replaced by DIN EN 24014 M6 x 30:8
- [Mate]: DIN 125-1 B B 6,4:8 ↔ DIN 931-1 - replaced by DIN EN 24014 M6 x 30:8
- [Mate]: DIN 125-1 B B 6,4:9 ↔ DIN 931-1 - replaced by DIN EN 24014 M6 x 30:9
- [Mate]: DIN 125-1 B B 6,4:9 ↔ DIN 931-1 - replaced by DIN EN 24014 M6 x 30:9
- [Mate]: DIN 125-1 B B 6,4:10 ↔ DIN 931-1 - replaced by DIN EN 24014 M6 x 30:10
- [Mate]: DIN 125-1 B B 6,4:10 ↔ DIN 931-1 - replaced by DIN EN 24014 M6 x 30:10
- [Mate]: DIN 125-1 B B 6,4:11 ↔ DIN 931-1 - replaced by DIN EN 24014 M6 x 30:11
- [Mate]: DIN 125-1 B B 6,4:11 ↔ DIN 931-1 - replaced by DIN EN 24014 M6 x 30:11
- [Mate]: DIN 125-1 B B 6,4:12 ↔ DIN 931-1 - replaced by DIN EN 24014 M6 x 30:12
- [Mate]: DIN 125-1 B B 6,4:12 ↔ DIN 931-1 - replaced by DIN EN 24014 M6 x 30:12
- [Mate]: DIN 125-1 B B 6,4:13 ↔ DIN 931-1 - replaced by DIN EN 24014 M6 x 30:13
- [Mate]: DIN 125-1 B B 6,4:13 ↔ DIN 931-1 - replaced by DIN EN 24014 M6 x 30:13
- [Mate]: DIN 125-1 B B 6,4:14 ↔ DIN 931-1 - replaced by DIN EN 24014 M6 x 30:14
- [Mate]: DIN 125-1 B B 6,4:14 ↔ DIN 931-1 - replaced by DIN EN 24014 M6 x 30:14
- [Mate]: DIN 125-1 B B 6,4:15 ↔ DIN 931-1 - replaced by DIN EN 24014 M6 x 30:15
- [Mate]: DIN 125-1 B B 6,4:15 ↔ DIN 931-1 - replaced by DIN EN 24014 M6 x 30:15
- [Mate]: DIN 125-1 B B 6,4:16 ↔ DIN 931-1 - replaced by DIN EN 24014 M6 x 30:16
- [Mate]: DIN 125-1 B B 6,4:16 ↔ DIN 931-1 - replaced by DIN EN 24014 M6 x 30:16
- [Mate]: DIN 125-1 B B 6,4:17 ↔ DIN 931-1 - replaced by DIN EN 24014 M6 x 30:17
- [Mate]: DIN 125-1 B B 6,4:17 ↔ DIN 931-1 - replaced by DIN EN 24014 M6 x 30:17
- [Mate]: DIN 125-1 B B 6,4:18 ↔ DIN 931-1 - replaced by DIN EN 24014 M6 x 30:18
- [Mate]: DIN 125-1 B B 6,4:18 ↔ DIN 931-1 - replaced by DIN EN 24014 M6 x 30:18
- [Mate]: DIN 125-1 B B 6,4:19 ↔ DIN 931-1 - replaced by DIN EN 24014 M6 x 30:19
- [Mate]: DIN 125-1 B B 6,4:19 ↔ DIN 931-1 - replaced by DIN EN 24014 M6 x 30:19
- [Mate]: DIN 125-1 B B 6,4:20 ↔ DIN 931-1 - replaced by DIN EN 24014 M6 x 30:20
- [Mate]: DIN 125-1 B B 6,4:20 ↔ DIN 931-1 - replaced by DIN EN 24014 M6 x 30:20
- Mate:191: Plattform-Oberteil:1 ↔ DIN 125-1 B B 6,4:19
- Mate:192: Plattform-Oberteil:1 ↔ DIN 125-1 B B 6,4:16
- Mate:193: Plattform-Oberteil:1 ↔ DIN 125-1 B B 6,4:20
- Mate:194: Plattform-Oberteil:1 ↔ DIN 125-1 B B 6,4:17
- Mate:195: Plattform-Oberteil:1 ↔ DIN 125-1 B B 6,4:10
- Mate:196: Plattform-Oberteil:1 ↔ DIN 125-1 B B 6,4:11
- Mate:197: Plattform-Oberteil:1 ↔ DIN 125-1 B B 6,4:4
- Mate:198: Plattform-Oberteil:1 ↔ DIN 125-1 B B 6,4:7
- Mate:199: Plattform-Oberteil:1 ↔ DIN 125-1 B B 6,4:18
- Mate:200: Plattform-Oberteil:1 ↔ DIN 125-1 B B 6,4:8
- Mate:201: Plattform-Oberteil:1 ↔ DIN 125-1 B B 6,4:13
- Mate:202: Plattform-Oberteil:1 ↔ DIN 125-1 B B 6,4:5
- Mate:203: Plattform-Oberteil:1 ↔ DIN 125-1 B B 6,4:15
- Mate:204: Plattform-Oberteil:1 ↔ DIN 125-1 B B 6,4:9
- Mate:205: Plattform-Oberteil:1 ↔ DIN 125-1 B B 6,4:14
- Mate:206: Plattform-Oberteil:1 ↔ DIN 125-1 B B 6,4:12
- Mate:207: Plattform-Oberteil:1 ↔ DIN 125-1 B B 6,4:17
- Mate:208: Federführungswellen:1 ↔ DIN 931-1 - replaced by DIN EN 24014 M6 x 30:19
- Mate:209: Federführungswellen:1 ↔ DIN 931-1 - replaced by DIN EN 24014 M6 x 30:20
- Mate:210: Federführungswellen:1 ↔ DIN 931-1 - replaced by DIN EN 24014 M6 x 30:16
- Mate:211: Federführungswellen:3 ↔ DIN 931-1 - replaced by DIN EN 24014 M6 x 30:11
- Mate:212: Federführungswellen:3 ↔ DIN 931-1 - replaced by DIN EN 24014 M6 x 30:4
- Mate:213: Federführungswellen:3 ↔ DIN 931-1 - replaced by DIN EN 24014 M6 x 30:10
- Mate:214: Federführungswellen:4 ↔ DIN 931-1 - replaced by DIN EN 24014 M6 x 30:8
- Mate:215: Federführungswellen:4 ↔ DIN 931-1 - replaced by DIN EN 24014 M6 x 30:7
- Mate:216: Federführungswellen:4 ↔ DIN 931-1 - replaced by DIN EN 24014 M6 x 30:18
- Mate:217: Federführungswellen:5 ↔ DIN 931-1 - replaced by DIN EN 24014 M6 x 30:5
- Mate:218: Federführungswellen:5 ↔ DIN 931-1 - replaced by DIN EN 24014 M6 x 30:13
- Mate:219: Federführungswellen:5 ↔ DIN 931-1 - replaced by DIN EN 24014 M6 x 30:15
- Mate:220: Federführungswellen:6 ↔ DIN 931-1 - replaced by DIN EN 24014 M6 x 30:9
- Mate:221: Federführungswellen:6 ↔ DIN 931-1 - replaced by DIN EN 24014 M6 x 30:14
- Mate:222: Federführungswellen:6 ↔ DIN 931-1 - replaced by DIN EN 24014 M6 x 30:12
- Mate:223: Plattform-Oberteil:1 ↔ DIN 931-1 - replaced by DIN EN 24014 M6 x 30:19